# Autodesk Inventor assembly: CAR_015_CarouselTensionerAssembly_MIR
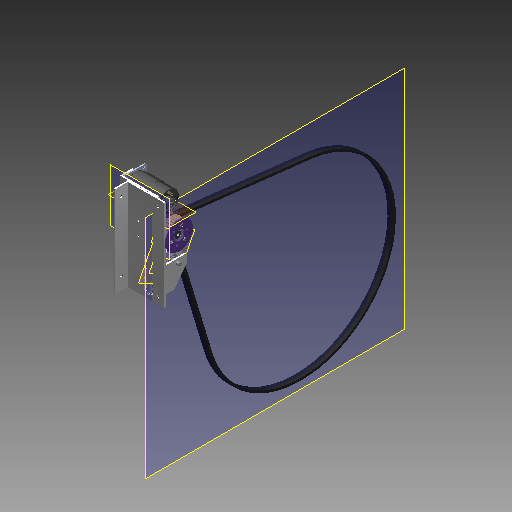
[picture p0: Inventor's stored thumbnail of the model, 512x512]
Saved by Autodesk Inventor 2018 (Build 220112000, 112)
## iProperties
Created: 2020-02-01
Part Number: CAR_015_CarouselTensionerAssembly_MIR
Document SubType Name: Assembly
Designer: user
Mass: 211.586 g
Surface Area: 527.901 cm^2
Volume: 81.806 cm^3
Density: 2.58644 g/cm^3
Author: user
## Documents named in this file (10)
- C:\Users\user\Documents\GrabCAD\New folder\Build season\CAR_015_CarouselTensionerAssembly_MIR.iam
- C:\Users\user\Documents\GrabCAD\New folder\Build season\CAR_014_CarouselTensionerPulley_MIR.ipt
- C:\Users\user\Documents\GrabCAD\New folder\Build season\CAR_016_TensionerMount_MIR.ipt
- C:\Users\user\Documents\GrabCAD\New folder\Build season\CAR_017_57155K305_STAINLESS STEEL BALL BEARING_MIR.ipt
- C:\Users\user\Documents\GrabCAD\New folder\Build season\CAR_018_98306A167_STEEL CLEVIS PIN_MIR.ipt
- C:\Users\user\Documents\GrabCAD\New folder\Build season\CAR_019_TensionerLBracket_MIR.ipt
- C:\Users\user\Documents\GrabCAD\New folder\Build season\CAR_020_217-3431_(CAM)_MIR.ipt
- C:\Users\user\Documents\GrabCAD\New folder\Build season\CAR_012_CarouselDriveAssembly.iam
- C:\Users\user\Documents\GrabCAD\New folder\Build season\CAR_033_CarouselBelt.ipt
- C:\Users\user\Documents\GrabCAD\New folder\Build season\CAR_044_180VersaLBracketMount.ipt
## Components (10 placed, 9 different names)
1. CAR_014_CarouselTensionerPulley_MIR:1 — Mate:3, Insert:1, Insert:2, Flush:2
2. CAR_016_TensionerMount_MIR:1 — Mate:3, Insert:3, Flush:1, Mate:2, Flush:3
3. CAR_017_57155K305_STAINLESS STEEL BALL BEARING_MIR:1 — Insert:1, Mate:1
4. CAR_017_57155K305_STAINLESS STEEL BALL BEARING_MIR:2 — Insert:2
5. CAR_018_98306A167_STEEL CLEVIS PIN_MIR:1 — Mate:1, Insert:3
6. CAR_019_TensionerLBracket_MIR:1 — Flush:1, Mate:2, Insert:4, Mate:5, Mate:6, Flush:3, Angle:1, Mate:9, Mate:10
7. CAR_020_217-3431_(CAM)_MIR:1 — Insert:4
8. CAR_012_CarouselDriveAssembly:1 [sub-assembly] — Mate:5, Mate:6, Mate:7, Mate:9, Mate:11, Flush:5
9. CAR_033_CarouselBelt:1 — Mate:7, Angle:1, Mate:8, Flush:4
10. CAR_044_180VersaLBracketMount:1 — Mate:10, Mate:11, Flush:5
## Relationships (20: Mate 10, Flush 5, Insert 4, Angle 1)
- Mate:3 (9.525 mm): CAR_014_CarouselTensionerPulley_MIR:1 ↔ CAR_016_TensionerMount_MIR:1
- Insert:1: CAR_014_CarouselTensionerPulley_MIR:1 ↔ CAR_017_57155K305_STAINLESS STEEL BALL BEARING_MIR:1
- Insert:2: CAR_014_CarouselTensionerPulley_MIR:1 ↔ CAR_017_57155K305_STAINLESS STEEL BALL BEARING_MIR:2
- Mate:1: CAR_017_57155K305_STAINLESS STEEL BALL BEARING_MIR:1 ↔ CAR_018_98306A167_STEEL CLEVIS PIN_MIR:1
- Insert:3: CAR_016_TensionerMount_MIR:1 ↔ CAR_018_98306A167_STEEL CLEVIS PIN_MIR:1
- Flush:1 (28.9052 mm): CAR_016_TensionerMount_MIR:1 ↔ CAR_019_TensionerLBracket_MIR:1
- Mate:2: CAR_016_TensionerMount_MIR:1 ↔ CAR_019_TensionerLBracket_MIR:1
- Insert:4: CAR_019_TensionerLBracket_MIR:1 ↔ CAR_020_217-3431_(CAM)_MIR:1
- Mate:5: CAR_019_TensionerLBracket_MIR:1 ↔ CAR_012_CarouselDriveAssembly:1
- Mate:6: CAR_019_TensionerLBracket_MIR:1 ↔ CAR_012_CarouselDriveAssembly:1
- Flush:2: CAR_014_CarouselTensionerPulley_MIR:1
- Flush:3 (19.05 mm): CAR_016_TensionerMount_MIR:1 ↔ CAR_019_TensionerLBracket_MIR:1
- Mate:7: CAR_012_CarouselDriveAssembly:1 ↔ CAR_033_CarouselBelt:1
- Angle:1 (0 deg): CAR_019_TensionerLBracket_MIR:1 ↔ CAR_033_CarouselBelt:1
- Mate:8: CAR_033_CarouselBelt:1
- Flush:4: CAR_033_CarouselBelt:1
- Mate:9 (3.175 mm): CAR_019_TensionerLBracket_MIR:1 ↔ CAR_012_CarouselDriveAssembly:1
- Mate:10: CAR_019_TensionerLBracket_MIR:1 ↔ CAR_044_180VersaLBracketMount:1
- Mate:11: CAR_012_CarouselDriveAssembly:1 ↔ CAR_044_180VersaLBracketMount:1
- Flush:5: CAR_012_CarouselDriveAssembly:1 ↔ CAR_044_180VersaLBracketMount:1
